# Autodesk Inventor assembly: fixfelsocsomopont
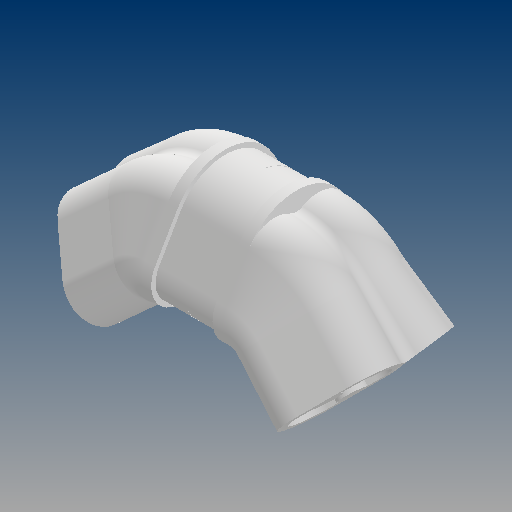
[picture p0: Inventor's stored thumbnail of the model, 512x512]
Saved by Autodesk Inventor 2023 (Build 270158000, 158)
## iProperties
Created: 2023-11-14
Part Number: fixfelsocsomopont
Document SubType Name: Assembly
Designer: gd1
Author: gd1
## Documents named in this file (2)
- C:\Users\gd1\3D Objects\Hid-main\Hid-main\new\hid2\felsocsomopont_fele_egesz.iam
- C:\Users\gd1\3D Objects\Hid-main\Hid-main\new\hid2\felsocsomopont_fele.ipt
## Components (2 placed, 1 different names)
1. felsocsomopont_fele:1 — Rigid:1
2. felsocsomopont_fele:2 — Rigid:1
## Relationships (1: WeldJoint 1)
- Rigid:1 [WeldJoint]: felsocsomopont_fele:1 ↔ felsocsomopont_fele:2
